# Autodesk Inventor assembly: Assembly1 kamera
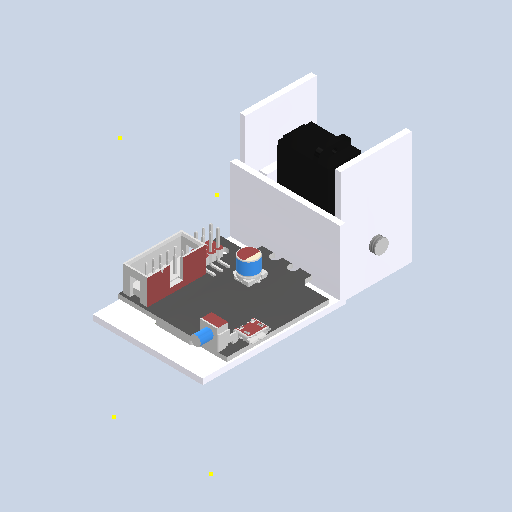
[picture p0: Inventor's stored thumbnail of the model, 512x512]
Saved by Autodesk Inventor 2023 (Build 270158000, 158)
## iProperties
Created: 2025-05-30
Part Number: Assembly1 kamera
Document SubType Name: Assembly
Designer: ASUS
Author: ASUS
## Documents named in this file (7)
- D:\Backup C\Documents\Inventor\PMLDCAPSTONE\fixasi\Assembly1 kamera.iam
- D:\Backup C\Documents\Inventor\PMLDCAPSTONE\fixasi\penyangga kamera 1.ipt
- D:\Backup C\Documents\Inventor\PMLDCAPSTONE\Servo EMAX ES08MDII.ipt
- D:\Backup C\Documents\Inventor\PMLDCAPSTONE\Peyangga Samping Kamera.ipt
- D:\Backup C\Documents\Inventor\PMLDCAPSTONE\Mur Kamera.ipt
- D:\Backup C\Documents\Inventor\PMLDCAPSTONE\fixasi\Kamera 2.ipt
- D:\Backup C\Documents\Inventor\PMLDCAPSTONE\pixy2\Pixy 2.ipt
## Components (8 placed, 6 different names)
1. penyangga kamera 1:1 — Mate:1, Mate:2, Mate:4
2. Servo EMAX ES08MDII:1 — Mate:1
3. Peyangga Samping Kamera:1 — Mate:5
4. Peyangga Samping Kamera:2 — Mate:3, Mate:6
5. Mur Kamera:1 — Mate:2, Mate:3
6. Mur Kamera:2 — Mate:4, Mate:5
7. Kamera 2:1 — Mate:6, Mate:7
8. Pixy 2:2 — Mate:7
## Relationships (7: Mate 7)
- Mate:1: penyangga kamera 1:1 ↔ Servo EMAX ES08MDII:1
- Mate:2: penyangga kamera 1:1 ↔ Mur Kamera:1
- Mate:3: Peyangga Samping Kamera:2 ↔ Mur Kamera:1
- Mate:4: penyangga kamera 1:1 ↔ Mur Kamera:2
- Mate:5: Peyangga Samping Kamera:1 ↔ Mur Kamera:2
- Mate:6: Peyangga Samping Kamera:2 ↔ Kamera 2:1
- Mate:7: Kamera 2:1 ↔ Pixy 2:2
